# Autodesk Inventor assembly: Prototype Assembly
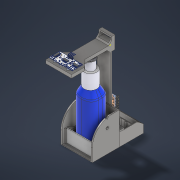
[picture p0: Inventor's stored thumbnail of the model, 180x180]
Saved by Autodesk Inventor 2022 (Build 260153000, 153)
## iProperties
Created: 2021-05-30
Part Number: Prototype Assembly
Document SubType Name: Assembly
Designer: sidsa
Author: sidsa
## Documents named in this file (10)
- D:\My Documents\gIThUB TWS\auto-dispenser\Inventor\Prototype Assembly.iam
- D:\My Documents\gIThUB TWS\auto-dispenser\Inventor\Hand Sanitizer (prototype).ipt
- D:\My Documents\gIThUB TWS\auto-dispenser\Inventor\PreCAD\ServoMotor.ipt
- D:\My Documents\gIThUB TWS\auto-dispenser\Inventor\Vertical Beam Prototype.ipt
- D:\My Documents\gIThUB TWS\auto-dispenser\Inventor\PreCAD\hc-sr04.ipt
- D:\My Documents\gIThUB TWS\auto-dispenser\Inventor\PreCAD\Arduino_NANO_CH340.ipt
- D:\My Documents\gIThUB TWS\auto-dispenser\Inventor\Base.ipt
- D:\My Documents\gIThUB TWS\auto-dispenser\Inventor\Sliding Plate.ipt
- D:\My Documents\gIThUB TWS\auto-dispenser\Inventor\Sliding Pin.ipt
- D:\My Documents\gIThUB TWS\auto-dispenser\Inventor\Electronics Tray.ipt
## Components (9 placed, 9 different names)
1. Hand Sanitizer (prototype):1 — Flush:4
2. ServoMotor:1 — Flush:6, Mate:9
3. Vertical Beam Prototype:1 — Flush:7, Mate:10, Mate:11, Mate:12, Mate:13, Mate:14, Mate:15
4. hc-sr04:1 — Mate:15
5. Arduino_NANO_CH340:1
6. Base:1 — Flush:4, Flush:5, Flush:6, Mate:9, Flush:7, Flush:8, Mate:10, Mate:11
7. Sliding Plate:1 — Flush:5
8. Sliding Pin:1 — Flush:8
9. Electronics Tray:1 — Mate:12, Mate:13, Mate:14
## Relationships (12: Mate 7, Flush 5)
- Flush:4: Hand Sanitizer (prototype):1 ↔ Base:1
- Flush:5: Base:1 ↔ Sliding Plate:1
- Flush:6: ServoMotor:1 ↔ Base:1
- Mate:9: ServoMotor:1 ↔ Base:1
- Flush:7: Vertical Beam Prototype:1 ↔ Base:1
- Flush:8: Base:1 ↔ Sliding Pin:1
- Mate:10: Vertical Beam Prototype:1 ↔ Base:1
- Mate:11: Vertical Beam Prototype:1 ↔ Base:1
- Mate:12: Vertical Beam Prototype:1 ↔ Electronics Tray:1
- Mate:13: Vertical Beam Prototype:1 ↔ Electronics Tray:1
- Mate:14: Vertical Beam Prototype:1 ↔ Electronics Tray:1
- Mate:15: Vertical Beam Prototype:1 ↔ hc-sr04:1
